# Autodesk Inventor assembly: roll축
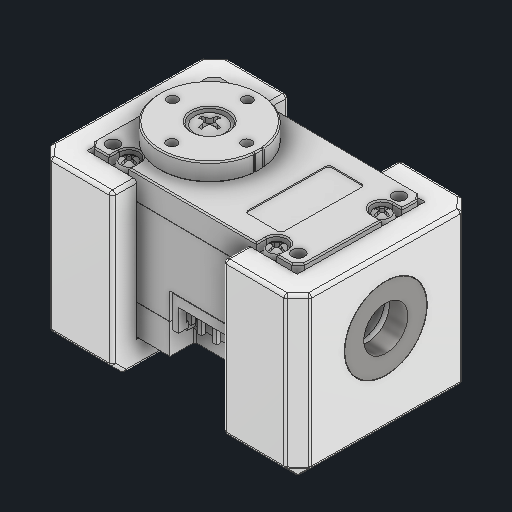
[picture p0: Inventor's stored thumbnail of the model, 512x512]
Saved by Autodesk Inventor 2027.1 (Build 311270010, 270A)
## iProperties
Created: 2026-08-10
Part Number: roll축
Document SubType Name: Assembly
Designer: moieboy9999
Mass: 33.5719 g
Surface Area: 175.321 cm^2
Volume: 25.1775 cm^3
Density: 1.33341 g/cm^3
Author: moieboy9999
## Documents named in this file (5)
- D:\micro_dog_cad\다리\프레임\roll축뒷다리.iam
- D:\micro_dog_cad\다리\프레임\롤프레임혼.ipt
- D:\micro_dog_cad\부품\XL,XC-330.ipt
- D:\micro_dog_cad\다리\프레임\롤프레임베어링.ipt
- D:\micro_dog_cad\부품\큰베어링.ipt
## Components (4 placed, 4 different names)
1. 롤프레임혼:1 — 메이트:13, 메이트:14, 메이트:15
2. 롤프레임베어링:1 — 메이트:11, 메이트:12, 메이트:16, 메이트:17
3. 큰베어링:1 — 메이트:11, 메이트:12, 메이트:13
4. XL,XC-330:1 — 메이트:14, 메이트:15, 메이트:16, 메이트:17
## Relationships (7: Mate 7)
- 메이트:11 [Mate]: 롤프레임베어링:1 ↔ 큰베어링:1
- 메이트:12 [Mate]: 롤프레임베어링:1 ↔ 큰베어링:1
- 메이트:13 [Mate]: 롤프레임혼:1 ↔ 큰베어링:1
- 메이트:14 [Mate]: 롤프레임혼:1 ↔ XL,XC-330:1
- 메이트:15 [Mate]: 롤프레임혼:1 ↔ XL,XC-330:1
- 메이트:16 [Mate]: 롤프레임베어링:1 ↔ XL,XC-330:1
- 메이트:17 [Mate]: 롤프레임베어링:1 ↔ XL,XC-330:1
